# Autodesk Inventor assembly: Carriage Assembly V1
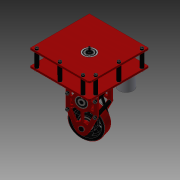
[picture p0: Inventor's stored thumbnail of the model, 180x180]
Saved by Autodesk Inventor 2013 (Build 170138000, 138)
## iProperties
Created: 2013-04-01
Part Number: Carriage Assembly V1
Document SubType Name: Assembly
Designer: mvarma
Author: mvarma
## Documents named in this file (11)
- C:\Users\mvarma\Desktop\Swerve Gearbox\Swerve Gearbox V1\Module Assembly V1.iam
- C:\Users\mvarma\Desktop\Swerve Gearbox\Swerve Gearbox V1\Module Plate - Bottom.ipt
- C:\Users\mvarma\Desktop\Swerve Gearbox\Swerve Gearbox V1\Imported Components\CIM Motor.ipt
- C:\Users\mvarma\Desktop\Swerve Gearbox\Swerve Gearbox V1\Banebots 550 Can - Temporary.ipt
- C:\Users\mvarma\Desktop\Swerve Gearbox\Swerve Gearbox V1\Module Plate - Top.ipt
- C:\Users\mvarma\Desktop\Swerve Gearbox\Swerve Gearbox V1\Imported Components\FR10-2RS.ipt
- C:\Users\mvarma\Desktop\Swerve Gearbox\Swerve Gearbox V1\Carriage Spacer - Thrust Bearing.ipt
- C:\Users\mvarma\Desktop\Swerve Gearbox\Swerve Gearbox V1\Module Standoff - Main.ipt
- C:\Users\mvarma\Desktop\Swerve Gearbox\Swerve Gearbox V1\Carriage Assembly V2 - Dead Axle.iam
- C:\Users\mvarma\Desktop\Swerve Gearbox\Swerve Gearbox V1\Imported Components\10-32 Thread Pem Nut.ipt
- C:\Users\mvarma\Desktop\Swerve Gearbox\Swerve Gearbox V1\Imported Components\Socket Head Cap Screw 10-32 Thread 2.000 Length.ipt
## Components (25 placed, 10 different names)
1. Module Plate - Bottom:1 — Angle:5, Mate:1, Mate:2, Mate:3, Mate:4, Flush:1, Flush:2, Mate:5, Mate:10, Mate:11, Mate:12, Mate:13, Mate:14, Mate:15, Mate:16, Mate:17, Mate:18, Mate:19, Mate:20, Mate:21, Mate:22, Mate:23, Mate:24, Mate:25, Mate:26, Mate:27, Mate:28, Mate:29, Mate:30, Mate:31, Mate:32, Mate:33
2. Carriage Assembly V2 - Dead Axle:1 [sub-assembly] — Mate:1, Mate:2
3. CIM Motor:1 — Mate:3
4. Banebots 550 Can - Temporary:1 — Mate:4
5. Module Plate - Top:1 — Flush:1, Flush:2, Mate:5, Mate:8, Mate:9, Mate:40, Mate:41, Mate:42, Mate:43, Mate:44, Mate:45
6. FR10-2RS:1 — Mate:6, Mate:7
7. Carriage Spacer - Thrust Bearing:1 — Mate:6, Mate:7, Mate:8, Mate:9
8. Module Standoff - Main:1 — Mate:10, Mate:20, Mate:34
9. Module Standoff - Main:2 — Mate:12, Mate:19, Mate:36
10. Module Standoff - Main:3 — Mate:11, Mate:21, Mate:35
11. Module Standoff - Main:4 — Mate:15, Mate:16, Mate:39
12. Module Standoff - Main:5 — Mate:14, Mate:17, Mate:38
13. Module Standoff - Main:6 — Mate:13, Mate:18, Mate:37
14. 10-32 Thread Pem Nut:1 — Mate:25, Mate:28
15. 10-32 Thread Pem Nut:2 — Mate:26, Mate:33
16. 10-32 Thread Pem Nut:3 — Mate:27, Mate:32
17. 10-32 Thread Pem Nut:4 — Mate:22, Mate:29
18. 10-32 Thread Pem Nut:5 — Mate:23, Mate:30
19. 10-32 Thread Pem Nut:6 — Mate:24, Mate:31
20. Socket Head Cap Screw 10-32 Thread 2.000 Length:1 — Mate:38, Mate:44
21. Socket Head Cap Screw 10-32 Thread 2.000 Length:2 — Mate:39, Mate:45
22. Socket Head Cap Screw 10-32 Thread 2.000 Length:3 — Mate:37, Mate:43
23. Socket Head Cap Screw 10-32 Thread 2.000 Length:4 — Mate:36, Mate:42
24. Socket Head Cap Screw 10-32 Thread 2.000 Length:5 — Mate:35, Mate:40
25. Socket Head Cap Screw 10-32 Thread 2.000 Length:6 — Mate:34, Mate:41
## Relationships (48: Mate 45, Flush 2, Angle 1)
- Angle:5 (0 deg): Module Plate - Bottom:1
- Mate:1: Module Plate - Bottom:1 ↔ Carriage Assembly V2 - Dead Axle:1
- Mate:2: Module Plate - Bottom:1 ↔ Carriage Assembly V2 - Dead Axle:1
- Mate:3: Module Plate - Bottom:1 ↔ CIM Motor:1
- Mate:4: Module Plate - Bottom:1 ↔ Banebots 550 Can - Temporary:1
- Flush:1: Module Plate - Bottom:1 ↔ Module Plate - Top:1
- Flush:2: Module Plate - Bottom:1 ↔ Module Plate - Top:1
- Mate:5 (38.1 mm): Module Plate - Bottom:1 ↔ Module Plate - Top:1
- Mate:6: FR10-2RS:1 ↔ Carriage Spacer - Thrust Bearing:1
- Mate:7: FR10-2RS:1 ↔ Carriage Spacer - Thrust Bearing:1
- Mate:8: Module Plate - Top:1 ↔ Carriage Spacer - Thrust Bearing:1
- Mate:9: Module Plate - Top:1 ↔ Carriage Spacer - Thrust Bearing:1
- Mate:10: Module Plate - Bottom:1 ↔ Module Standoff - Main:1
- Mate:11: Module Plate - Bottom:1 ↔ Module Standoff - Main:3
- Mate:12: Module Plate - Bottom:1 ↔ Module Standoff - Main:2
- Mate:13: Module Plate - Bottom:1 ↔ Module Standoff - Main:6
- Mate:14: Module Plate - Bottom:1 ↔ Module Standoff - Main:5
- Mate:15: Module Plate - Bottom:1 ↔ Module Standoff - Main:4
- Mate:16: Module Plate - Bottom:1 ↔ Module Standoff - Main:4
- Mate:17: Module Plate - Bottom:1 ↔ Module Standoff - Main:5
- Mate:18: Module Plate - Bottom:1 ↔ Module Standoff - Main:6
- Mate:19: Module Plate - Bottom:1 ↔ Module Standoff - Main:2
- Mate:20: Module Plate - Bottom:1 ↔ Module Standoff - Main:1
- Mate:21: Module Plate - Bottom:1 ↔ Module Standoff - Main:3
- Mate:22: Module Plate - Bottom:1 ↔ 10-32 Thread Pem Nut:4
- Mate:23: Module Plate - Bottom:1 ↔ 10-32 Thread Pem Nut:5
- Mate:24: Module Plate - Bottom:1 ↔ 10-32 Thread Pem Nut:6
- Mate:25: Module Plate - Bottom:1 ↔ 10-32 Thread Pem Nut:1
- Mate:26: Module Plate - Bottom:1 ↔ 10-32 Thread Pem Nut:2
- Mate:27: Module Plate - Bottom:1 ↔ 10-32 Thread Pem Nut:3
- Mate:28: Module Plate - Bottom:1 ↔ 10-32 Thread Pem Nut:1
- Mate:29: Module Plate - Bottom:1 ↔ 10-32 Thread Pem Nut:4
- Mate:30: Module Plate - Bottom:1 ↔ 10-32 Thread Pem Nut:5
- Mate:31: Module Plate - Bottom:1 ↔ 10-32 Thread Pem Nut:6
- Mate:32: Module Plate - Bottom:1 ↔ 10-32 Thread Pem Nut:3
- Mate:33: Module Plate - Bottom:1 ↔ 10-32 Thread Pem Nut:2
- Mate:34: Module Standoff - Main:1 ↔ Socket Head Cap Screw 10-32 Thread 2.000 Length:6
- Mate:35: Module Standoff - Main:3 ↔ Socket Head Cap Screw 10-32 Thread 2.000 Length:5
- Mate:36: Module Standoff - Main:2 ↔ Socket Head Cap Screw 10-32 Thread 2.000 Length:4
- Mate:37: Module Standoff - Main:6 ↔ Socket Head Cap Screw 10-32 Thread 2.000 Length:3
- Mate:38: Module Standoff - Main:5 ↔ Socket Head Cap Screw 10-32 Thread 2.000 Length:1
- Mate:39: Module Standoff - Main:4 ↔ Socket Head Cap Screw 10-32 Thread 2.000 Length:2
- Mate:40: Module Plate - Top:1 ↔ Socket Head Cap Screw 10-32 Thread 2.000 Length:5
- Mate:41: Module Plate - Top:1 ↔ Socket Head Cap Screw 10-32 Thread 2.000 Length:6
- Mate:42: Module Plate - Top:1 ↔ Socket Head Cap Screw 10-32 Thread 2.000 Length:4
- Mate:43: Module Plate - Top:1 ↔ Socket Head Cap Screw 10-32 Thread 2.000 Length:3
- Mate:44: Module Plate - Top:1 ↔ Socket Head Cap Screw 10-32 Thread 2.000 Length:1
- Mate:45: Module Plate - Top:1 ↔ Socket Head Cap Screw 10-32 Thread 2.000 Length:2
## Named parameters: x = 0 deg
